# Autodesk Inventor assembly: B3OFT4_HF2_kezifuro_Assembly.ipt
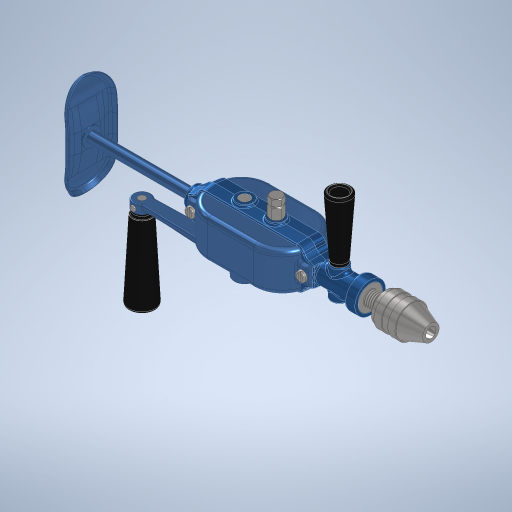
[picture p0: Inventor's stored thumbnail of the model, 512x512]
Saved by Autodesk Inventor 2023.3 (Build 273359000, 359)
## iProperties
Created: 2023-11-22
Part Number: B3OFT4_HF2_kezifuro_Assembly.ipt
Document SubType Name: Assembly
Designer: Csábi-Kis Henrik
Mass: 1532.95 g
Surface Area: 1311.83 cm^2
Volume: 210.513 cm^3
Density: 7.28197 g/cm^3
Author: Csábi-Kis Henrik
## Documents named in this file (21)
- C:\Users\cskhe\OneDrive\Documents\Egyetem\V. felev\CAD modellezes\HF2\B3OFT4_HF2_kezifuro_Assembly.iam
- C:\Users\cskhe\OneDrive\Documents\Egyetem\V. felev\CAD modellezes\HF2\B3OFT4_HF2_kezifuro_skeleton.ipt
- C:\Users\cskhe\OneDrive\Documents\Egyetem\V. felev\CAD modellezes\HF2\B3OFT4_HF2_kezifuro_EgyenesFogaskerekTengely.ipt
- C:\Users\cskhe\OneDrive\Documents\Egyetem\V. felev\CAD modellezes\HF2\B3OFT4_HF2_kezifuro_NagyKupFogaskerekTengely.ipt
- C:\Users\cskhe\OneDrive\Documents\Egyetem\V. felev\CAD modellezes\HF2\B3OFT4_HF2_kezifuro_TokmanyTengely.ipt
- C:\Users\cskhe\OneDrive\Documents\Egyetem\V. felev\CAD modellezes\HF2\B3OFT4_HF2_kezifuro_Haz.ipt
- C:\Users\cskhe\OneDrive\Documents\Egyetem\V. felev\CAD modellezes\HF2\B3OFT4_HF2_kezifuro_Assembly\Design Accelerator\Spur Gears1.iam
- C:\Users\cskhe\OneDrive\Documents\Egyetem\V. felev\CAD modellezes\HF2\B3OFT4_HF2_kezifuro_Assembly\Design Accelerator\Bevel Gears1.iam
- C:\Users\cskhe\OneDrive\Documents\Egyetem\V. felev\CAD modellezes\HF2\Csapagy.iam
- C:\Users\cskhe\OneDrive\Documents\Egyetem\V. felev\CAD modellezes\HF2\B3OFT4_HF2_kezifuro_Tamaszto.ipt
- C:\Users\cskhe\OneDrive\Documents\Egyetem\V. felev\CAD modellezes\HF2\ISO 2338 - 3 h11 x 20 - C(2).ipt
- C:\Users\cskhe\OneDrive\Documents\Egyetem\V. felev\CAD modellezes\HF2\ISO 2338 - 3 h11 x 16 - C(2).ipt
- C:\Users\cskhe\OneDrive\Documents\Egyetem\V. felev\CAD modellezes\HF2\B3OFT4_HF2_kezifuro_Tokmany.ipt
- C:\Users\cskhe\OneDrive\Documents\Egyetem\V. felev\CAD modellezes\HF2\B3OFT4_HF2_kezifuro_Hajtokar.ipt
- C:\Users\cskhe\OneDrive\Documents\Egyetem\V. felev\CAD modellezes\HF2\B3OFT4_HF2_kezifuro_NagySzegecs.ipt
- C:\Users\cskhe\OneDrive\Documents\Egyetem\V. felev\CAD modellezes\HF2\ISO_R 1051 - 3 x 25 x 17.ipt
- C:\Users\cskhe\OneDrive\Documents\Egyetem\V. felev\CAD modellezes\HF2\B3OFT4_HF2_kezifuro_HajtokarFogo.ipt
- C:\Users\cskhe\OneDrive\Documents\Egyetem\V. felev\CAD modellezes\HF2\B3OFT4_HF2_kezifuro_Fogo.ipt
- C:\Users\cskhe\OneDrive\Documents\Egyetem\V. felev\CAD modellezes\HF2\B3OFT4_HF2_kezifuro_HajtokarCsavar.ipt
- C:\Users\cskhe\OneDrive\Documents\Egyetem\V. felev\CAD modellezes\HF2\B3OFT4_HF2_kezifuro_Fedo.ipt
- C:\Users\cskhe\OneDrive\Documents\Egyetem\V. felev\CAD modellezes\HF2\ISO 1580 - M5 x 8_.ipt
## Components (25 placed, 20 different names)
1. B3OFT4_HF2_kezifuro_skeleton:1 — Flush:1, Flush:2, Flush:3, Mate:59, Mate:61, Angle:15, Angle:16
2. B3OFT4_HF2_kezifuro_EgyenesFogaskerekTengely:1 — Insert:1, Mate:10, Mate:35, Mate:36, Angle:8, Mate:44, Mate:45, Tangent:1, Mate:58
3. B3OFT4_HF2_kezifuro_NagyKupFogaskerekTengely:1 — Insert:2, Mate:15, Angle:3, Mate:33, Mate:34, Angle:7, Mate:60, Mate:62
4. B3OFT4_HF2_kezifuro_TokmanyTengely:1 — Insert:3, Angle:6, Mate:28, Mate:30, Mate:31, Mate:32, Insert:5, Mate:63
5. B3OFT4_HF2_kezifuro_Haz:1 — Flush:11, Flush:12, Flush:13, Insert:1, Insert:2, Insert:3, Flush:14, Insert:4, Insert:8, Mate:57
6. Spur Gears:1 [sub-assembly] — Mate:10, Mate:15, Mate:58, Mate:59, Mate:60, Mate:61
7. Bevel Gears:1 [sub-assembly] — Angle:3, Angle:6, Mate:62, Angle:15, Mate:63, Angle:16
8. Csapagy:1 [sub-assembly] — Mate:28, Flush:14, Mate:37
9. B3OFT4_HF2_kezifuro_Tamaszto:1 — Insert:4
10. ISO 2338 C - withdrawn 3 h11 x 20 - C:1 — Mate:35, Mate:36, Angle:8
11. ISO 2338 C - withdrawn 3 h11 x 20 - C:2 — Mate:33, Mate:34, Angle:7
12. ISO 2338 C - withdrawn 3 h11 x 16 - C:1 — Mate:30, Mate:31, Mate:32
13. B3OFT4_HF2_kezifuro_Tokmany:1 — Insert:5
14. B3OFT4_HF2_kezifuro_Hajtokar:1 — Flush:15, Mate:44, Mate:45, Insert:6, Angle:11, Mate:47, Mate:54
15. B3OFT4_HF2_kezifuro_NagySzegecs:1 — Insert:6, Mate:46, Insert:7
16. ISO_R 1051 - 3 x 25 x 17:1 — Mate:46, Angle:11, Mate:47
17. B3OFT4_HF2_kezifuro_HajtokarFogo:1 — Insert:7
18. B3OFT4_HF2_kezifuro_Fogo:1 — Insert:8
19. B3OFT4_HF2_kezifuro_HajtokarCsavar:1 — Angle:14, Mate:54, Tangent:1
20. B3OFT4_HF2_kezifuro_Fedo:1 — Flush:16, Mate:55, Mate:56, Insert:11, Insert:12
21. B3OFT4_HF2_kezifuro_Fedo:2 — Flush:17, Flush:18, Mate:57, Insert:9, Insert:10
22. ISO 1580 M5 x 8:1 — Insert:9
23. ISO 1580 M5 x 8:2 — Insert:10
24. ISO 1580 M5 x 8:3 — Insert:11
25. ISO 1580 M5 x 8:4 — Insert:12
## Relationships (57: Mate 25, Insert 12, Flush 11, Angle 8, Tangent 1)
- Flush:1: B3OFT4_HF2_kezifuro_skeleton:1
- Flush:2: B3OFT4_HF2_kezifuro_skeleton:1
- Flush:3: B3OFT4_HF2_kezifuro_skeleton:1
- Flush:11: B3OFT4_HF2_kezifuro_Haz:1
- Flush:12: B3OFT4_HF2_kezifuro_Haz:1
- Flush:13: B3OFT4_HF2_kezifuro_Haz:1
- Insert:1: B3OFT4_HF2_kezifuro_EgyenesFogaskerekTengely:1 ↔ B3OFT4_HF2_kezifuro_Haz:1
- Mate:10: B3OFT4_HF2_kezifuro_EgyenesFogaskerekTengely:1 ↔ Spur Gears:1
- Insert:2: B3OFT4_HF2_kezifuro_NagyKupFogaskerekTengely:1 ↔ B3OFT4_HF2_kezifuro_Haz:1
- Mate:15: B3OFT4_HF2_kezifuro_NagyKupFogaskerekTengely:1 ↔ Spur Gears:1
- Angle:3 (0 deg): B3OFT4_HF2_kezifuro_NagyKupFogaskerekTengely:1 ↔ Bevel Gears:1
- Insert:3: B3OFT4_HF2_kezifuro_TokmanyTengely:1 ↔ B3OFT4_HF2_kezifuro_Haz:1
- Angle:6 (0 deg): B3OFT4_HF2_kezifuro_TokmanyTengely:1 ↔ Bevel Gears:1
- Mate:28: B3OFT4_HF2_kezifuro_TokmanyTengely:1 ↔ Csapagy:1
- Flush:14: B3OFT4_HF2_kezifuro_Haz:1 ↔ Csapagy:1
- Insert:4: B3OFT4_HF2_kezifuro_Haz:1 ↔ B3OFT4_HF2_kezifuro_Tamaszto:1
- Mate:30: B3OFT4_HF2_kezifuro_TokmanyTengely:1 ↔ ISO 2338 C - withdrawn 3 h11 x 16 - C:1
- Mate:31 (8 mm): B3OFT4_HF2_kezifuro_TokmanyTengely:1 ↔ ISO 2338 C - withdrawn 3 h11 x 16 - C:1
- Mate:32: B3OFT4_HF2_kezifuro_TokmanyTengely:1 ↔ ISO 2338 C - withdrawn 3 h11 x 16 - C:1
- Mate:33 (10 mm): B3OFT4_HF2_kezifuro_NagyKupFogaskerekTengely:1 ↔ ISO 2338 C - withdrawn 3 h11 x 20 - C:2
- Mate:34: B3OFT4_HF2_kezifuro_NagyKupFogaskerekTengely:1 ↔ ISO 2338 C - withdrawn 3 h11 x 20 - C:2
- Angle:7 (0 deg): B3OFT4_HF2_kezifuro_NagyKupFogaskerekTengely:1 ↔ ISO 2338 C - withdrawn 3 h11 x 20 - C:2
- Mate:35 (10 mm): B3OFT4_HF2_kezifuro_EgyenesFogaskerekTengely:1 ↔ ISO 2338 C - withdrawn 3 h11 x 20 - C:1
- Mate:36: B3OFT4_HF2_kezifuro_EgyenesFogaskerekTengely:1 ↔ ISO 2338 C - withdrawn 3 h11 x 20 - C:1
- Angle:8 (0 deg): B3OFT4_HF2_kezifuro_EgyenesFogaskerekTengely:1 ↔ ISO 2338 C - withdrawn 3 h11 x 20 - C:1
- Insert:5 (-15 mm): B3OFT4_HF2_kezifuro_TokmanyTengely:1 ↔ B3OFT4_HF2_kezifuro_Tokmany:1
- Mate:37: Csapagy:1
- Flush:15: B3OFT4_HF2_kezifuro_Hajtokar:1
- Mate:44: B3OFT4_HF2_kezifuro_EgyenesFogaskerekTengely:1 ↔ B3OFT4_HF2_kezifuro_Hajtokar:1
- Mate:45: B3OFT4_HF2_kezifuro_EgyenesFogaskerekTengely:1 ↔ B3OFT4_HF2_kezifuro_Hajtokar:1
- Insert:6: B3OFT4_HF2_kezifuro_Hajtokar:1 ↔ B3OFT4_HF2_kezifuro_NagySzegecs:1
- Mate:46: B3OFT4_HF2_kezifuro_NagySzegecs:1 ↔ ISO_R 1051 - 3 x 25 x 17:1
- Angle:11 (0 deg): B3OFT4_HF2_kezifuro_Hajtokar:1 ↔ ISO_R 1051 - 3 x 25 x 17:1
- Mate:47 (8.5 mm): B3OFT4_HF2_kezifuro_Hajtokar:1 ↔ ISO_R 1051 - 3 x 25 x 17:1
- Insert:7: B3OFT4_HF2_kezifuro_NagySzegecs:1 ↔ B3OFT4_HF2_kezifuro_HajtokarFogo:1
- Insert:8: B3OFT4_HF2_kezifuro_Haz:1 ↔ B3OFT4_HF2_kezifuro_Fogo:1
- Angle:14 (0 deg): B3OFT4_HF2_kezifuro_HajtokarCsavar:1
- Mate:54: B3OFT4_HF2_kezifuro_Hajtokar:1 ↔ B3OFT4_HF2_kezifuro_HajtokarCsavar:1
- Tangent:1: B3OFT4_HF2_kezifuro_EgyenesFogaskerekTengely:1 ↔ B3OFT4_HF2_kezifuro_HajtokarCsavar:1
- Flush:16: B3OFT4_HF2_kezifuro_Fedo:1
- Mate:55: B3OFT4_HF2_kezifuro_Fedo:1
- Mate:56: B3OFT4_HF2_kezifuro_Fedo:1
- Flush:17: B3OFT4_HF2_kezifuro_Fedo:2
- Flush:18: B3OFT4_HF2_kezifuro_Fedo:2
- Mate:57: B3OFT4_HF2_kezifuro_Haz:1 ↔ B3OFT4_HF2_kezifuro_Fedo:2
- Insert:9: B3OFT4_HF2_kezifuro_Fedo:2 ↔ ISO 1580 M5 x 8:1
- Insert:10: B3OFT4_HF2_kezifuro_Fedo:2 ↔ ISO 1580 M5 x 8:2
- Insert:11: B3OFT4_HF2_kezifuro_Fedo:1 ↔ ISO 1580 M5 x 8:3
- Insert:12: B3OFT4_HF2_kezifuro_Fedo:1 ↔ ISO 1580 M5 x 8:4
- Mate:58: B3OFT4_HF2_kezifuro_EgyenesFogaskerekTengely:1 ↔ Spur Gears:1
- Mate:59: B3OFT4_HF2_kezifuro_skeleton:1 ↔ Spur Gears:1
- Mate:60: B3OFT4_HF2_kezifuro_NagyKupFogaskerekTengely:1 ↔ Spur Gears:1
- Mate:61: B3OFT4_HF2_kezifuro_skeleton:1 ↔ Spur Gears:1
- Mate:62: B3OFT4_HF2_kezifuro_NagyKupFogaskerekTengely:1 ↔ Bevel Gears:1
- Angle:15 (0 deg): B3OFT4_HF2_kezifuro_skeleton:1 ↔ Bevel Gears:1
- Mate:63: B3OFT4_HF2_kezifuro_TokmanyTengely:1 ↔ Bevel Gears:1
- Angle:16 (0 deg): B3OFT4_HF2_kezifuro_skeleton:1 ↔ Bevel Gears:1
## Named parameters: HazBelsoSzelesseg = 30 mm, HazBelsoHosszusag = 87 mm, HazFalVastagsag = 6 mm, HazMagassag = 22 mm, FedolemezMagassag = 19.8 mm, FogaskerekTengelyAtmero = 10 mm, BelsoFelfekvesTavolsag = -27.5 mm, FogaskerekTengelyVallMagassag = -48 mm, FogaskerekTengelyHossz = -66 mm, FogaskerekTengelyLapTavolsag = 11 mm, TamasztoMenet = 10 mm, FedolemezCsavarAtmero = 5 mm, FedolemezCsavarTavolsag = 108 mm, TengelyTavolsag = 30.8 mm, TengelyOffset = 29.4 mm, FuroTengelyAtmero = 10 mm, CsapagyFogoOffset = 63 mm, CsapagyKulsoAtmero = 24 mm, CsapagyFogoMelyseg = -6 mm, TokmanyMenet = 14 mm, SzegAtmero = 3 mm, EgyenesTengelySzegTavolsag = 20.5 mm, NagyKupTengelySzegTavolsag = 28.5 mm, FogoMenet = 8 mm, FogoTavolsag = 30 mm, TamasztoHossz = 100 mm, HajtkarClearance = 2 mm, HajtokarNagyAtmero = 23 mm, HajtokarHossz = 100 mm, HajtokarKisAtmero = 17 mm, HajtokarKisMagassag = 9 mm, HajtokarSzegAtmero = 7 mm, HajtokarSzegHossz = 45 mm, HajtokarFogoBelsoAtmero = 14 mm, HajtokarCsavarMenet = 6 mm, HajtokarCsavarTavolsag = 7 mm, FogaskerekFelfekvesOffset = 1 mm, EgyenesFogasKerekSzelesseg = 12 mm, KisKupkerekFogOffset = -5.5 mm, KupkerekBelsoCsatlakozas = 13 mm, FogaskerekTengelyHatszogHossz = 18 mm, NagySzegHossz = 20 mm, KisSzegHossz = 16 mm
